# Autodesk Inventor assembly: propeler + motor
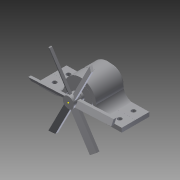
[picture p0: Inventor's stored thumbnail of the model, 180x180]
Saved by Autodesk Inventor 2012 (Build 160160000, 160)
## iProperties
Created: 2012-12-20
Part Number: propeler + motor
Document SubType Name: Assembly
Designer: Irwan Haryanto
Author: Irwan Haryanto
## Documents named in this file (4)
- D:\TRUI Ruby\propeler + motor.iam
- D:\TRUI Ruby\motor kipas.ipt
- D:\TRUI Ruby\propeler.ipt
- D:\TRUI Ruby\braket motor kipas.ipt
## Components (4 placed, 3 different names)
1. motor kipas:1 — Insert:1, Mate:4, Mate:5
2. propeler:1 — Insert:1
3. braket motor kipas:1 — Mate:1, Mate:2, Mate:3, Mate:4, Mate:5
4. braket motor kipas:2 — Mate:1, Mate:2, Mate:3
## Relationships (6: Mate 5, Insert 1)
- Insert:1: motor kipas:1 ↔ propeler:1
- Mate:1: braket motor kipas:1 ↔ braket motor kipas:2
- Mate:2: braket motor kipas:1 ↔ braket motor kipas:2
- Mate:3: braket motor kipas:1 ↔ braket motor kipas:2
- Mate:4: motor kipas:1 ↔ braket motor kipas:1
- Mate:5: motor kipas:1 ↔ braket motor kipas:1
